# Autodesk Inventor assembly: mg996r 3mm middle base leg
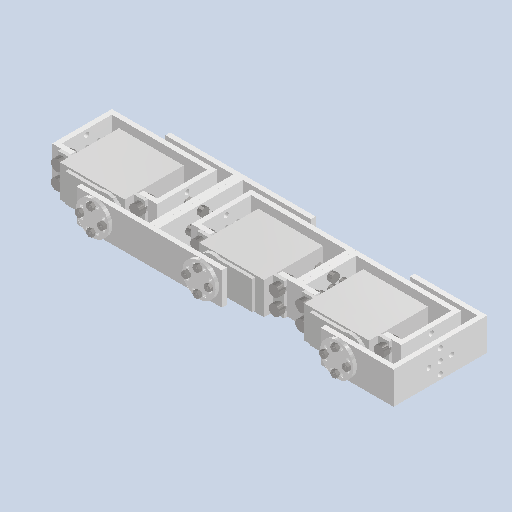
[picture p0: Inventor's stored thumbnail of the model, 512x512]
Saved by Autodesk Inventor 2023 (Build 270158000, 158)
## iProperties
Created: 2022-06-29
Part Number: mg996r 3mm middle base leg
Document SubType Name: Assembly
Designer: isamu
Author: isamu
## Documents named in this file (4)
- D:\personal_projects\robot\inventor\mg996r 3mm middle base leg.iam
- D:\personal_projects\robot\inventor\mg996r 3mm middle base.iam
- D:\personal_projects\robot\exports\frames\m3x8.ipt
- D:\personal_projects\robot\exports\frames\m3 nuts.ipt
## Components (23 placed, 3 different names)
1. mg996r 3mm middle base:1 [sub-assembly] — Mate:1, Mate:2, Mate:3, Insert:16, Insert:17, Insert:18, Insert:19, Insert:20
2. mg996r 3mm middle base:2 [sub-assembly] — Mate:1, Mate:2, Mate:3, Mate:4, Mate:5, Mate:6, Insert:1, Insert:2, Insert:3, Insert:4, Insert:5, Insert:11, Insert:12, Insert:13, Insert:14, Insert:15
3. mg996r 3mm middle base:3 [sub-assembly] — Mate:4, Mate:5, Mate:6, Insert:6, Insert:7, Insert:8, Insert:9, Insert:10
4. m3x8:1 — Insert:2
5. m3x8:2 — Insert:6
6. m3x8:3 — Insert:9
7. m3x8:4 — Insert:10
8. m3x8:5 — Insert:3
9. m3x8:6 — Insert:1
10. m3x8:7 — Insert:4
11. m3x8:8 — Insert:5
12. m3x8:9 — Insert:8
13. m3x8:10 — Insert:7
14. m3 nuts:1 — Insert:11
15. m3 nuts:2 — Insert:12
16. m3 nuts:3 — Insert:13
17. m3 nuts:4 — Insert:14
18. m3 nuts:5 — Insert:15
19. m3 nuts:6 — Insert:16
20. m3 nuts:7 — Insert:17
21. m3 nuts:8 — Insert:18
22. m3 nuts:9 — Insert:19
23. m3 nuts:10 — Insert:20
## Relationships (26: Insert 20, Mate 6)
- Mate:1: mg996r 3mm middle base:1 ↔ mg996r 3mm middle base:2
- Mate:2: mg996r 3mm middle base:1 ↔ mg996r 3mm middle base:2
- Mate:3: mg996r 3mm middle base:1 ↔ mg996r 3mm middle base:2
- Mate:4: mg996r 3mm middle base:2 ↔ mg996r 3mm middle base:3
- Mate:5: mg996r 3mm middle base:2 ↔ mg996r 3mm middle base:3
- Mate:6: mg996r 3mm middle base:2 ↔ mg996r 3mm middle base:3
- Insert:1: mg996r 3mm middle base:2 ↔ m3x8:6
- Insert:2: mg996r 3mm middle base:2 ↔ m3x8:1
- Insert:3: mg996r 3mm middle base:2 ↔ m3x8:5
- Insert:4: mg996r 3mm middle base:2 ↔ m3x8:7
- Insert:5: mg996r 3mm middle base:2 ↔ m3x8:8
- Insert:6: mg996r 3mm middle base:3 ↔ m3x8:2
- Insert:7: mg996r 3mm middle base:3 ↔ m3x8:10
- Insert:8: mg996r 3mm middle base:3 ↔ m3x8:9
- Insert:9: mg996r 3mm middle base:3 ↔ m3x8:3
- Insert:10: mg996r 3mm middle base:3 ↔ m3x8:4
- Insert:11: mg996r 3mm middle base:2 ↔ m3 nuts:1
- Insert:12: mg996r 3mm middle base:2 ↔ m3 nuts:2
- Insert:13: mg996r 3mm middle base:2 ↔ m3 nuts:3
- Insert:14: mg996r 3mm middle base:2 ↔ m3 nuts:4
- Insert:15: mg996r 3mm middle base:2 ↔ m3 nuts:5
- Insert:16: mg996r 3mm middle base:1 ↔ m3 nuts:6
- Insert:17: mg996r 3mm middle base:1 ↔ m3 nuts:7
- Insert:18: mg996r 3mm middle base:1 ↔ m3 nuts:8
- Insert:19: mg996r 3mm middle base:1 ↔ m3 nuts:9
- Insert:20: mg996r 3mm middle base:1 ↔ m3 nuts:10
